# Autodesk Inventor assembly: Ensemble_Lanceur
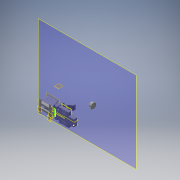
[picture p0: Inventor's stored thumbnail of the model, 180x180]
Saved by Autodesk Inventor 2017 (Build 210142000, 142)
## iProperties
Part Number: Ensemble_Lanceur
Material: Générique
Document SubType Name: Assembly
Designer: Thomas
Author: Thomas
## Documents named in this file (12)
- C:\Users\Thomas\Documents\Modele 3D\Lanceur boule\Ensemble_Lanceur.iam
- C:\Users\Thomas\Documents\Modele 3D\Lanceur boule\cremaillere.ipt
- C:\Users\Thomas\Documents\Modele 3D\Lanceur boule\lanceur.ipt
- C:\Users\Thomas\Documents\Modele 3D\Lanceur boule\Ensemble_Lanceur\Design Accelerator\Engrenages cylindriques4.iam
- C:\Users\Thomas\Documents\Modele 3D\Lanceur boule\support_arret.ipt
- C:\Users\Thomas\Documents\Modele 3D\Lanceur boule\aret.ipt
- C:\Users\Thomas\Documents\Modele 3D\Lanceur boule\percuteur.ipt
- C:\Users\Thomas\Documents\Modele 3D\Lanceur boule\new_cuiller.ipt
- C:\Users\Thomas\Documents\Modele 3D\Lanceur boule\enclenchement.ipt
- C:\Users\Thomas\Documents\Modele 3D\Lanceur boule\courbe.ipt
- C:\Users\Thomas\Documents\Modele 3D\Lanceur boule\tg.ipt
- C:\Users\Thomas\Documents\Modele 3D\Lanceur boule\Boule.ipt
## Components (11 placed, 11 different names)
1. cremaillere:1 — Placage:17, Placage:18, Placage:19, Placage:20
2. lanceur:1 — Placage:10, Placage:12, Placage:13, Placage:14, Placage:17, Affleurement:7
3. Engrenages cylindriques:2 [sub-assembly]
4. aret:1 — Placage:14, Placage:15, Affleurement:1, Placage:18, Affleurement:3, Affleurement:4, Affleurement:5, Affleurement:6
5. support_arret:1 — Placage:11, Placage:12, Placage:13, Placage:15, Affleurement:1
6. percuteur:1 — Placage:19, Placage:20
7. new_cuiller:1 — Affleurement:7, Placage:28
8. enclenchement:1 — Affleurement:3, Placage:24, Placage:27
9. courbe:1 — Placage:24, Placage:27
10. tg:1 — Affleurement:5, Affleurement:6
11. Boule:1 — Placage:28
## Relationships (19: Mate 13, Flush 6)
- Placage:10 [Mate]: lanceur:1
- Placage:11 [Mate]: support_arret:1
- Placage:12 [Mate]: lanceur:1 ↔ support_arret:1
- Placage:13 [Mate]: lanceur:1 ↔ support_arret:1
- Placage:14 [Mate]: lanceur:1 ↔ aret:1
- Placage:15 [Mate]: aret:1 ↔ support_arret:1
- Affleurement:1 [Flush]: aret:1 ↔ support_arret:1
- Placage:17 [Mate]: cremaillere:1 ↔ lanceur:1
- Placage:18 [Mate]: cremaillere:1 ↔ aret:1
- Placage:19 [Mate]: cremaillere:1 ↔ percuteur:1
- Placage:20 [Mate]: cremaillere:1 ↔ percuteur:1
- Affleurement:3 [Flush]: aret:1 ↔ enclenchement:1
- Affleurement:4 [Flush] (100 mm): aret:1
- Placage:24 [Mate]: enclenchement:1 ↔ courbe:1
- Placage:27 [Mate]: enclenchement:1 ↔ courbe:1
- Affleurement:5 [Flush]: aret:1 ↔ tg:1
- Affleurement:6 [Flush]: aret:1 ↔ tg:1
- Affleurement:7 [Flush] (15 mm): lanceur:1 ↔ new_cuiller:1
- Placage:28 [Mate] (24.5 mm): new_cuiller:1 ↔ Boule:1
